# Autodesk Inventor assembly: MGN12H_With_Rail
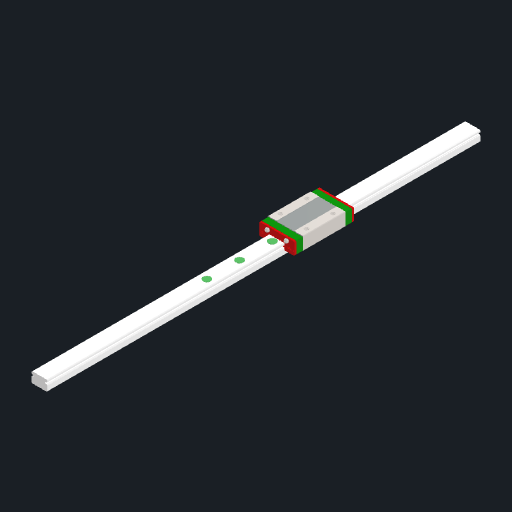
[picture p0: Inventor's stored thumbnail of the model, 512x512]
Saved by Autodesk Inventor 2026.2 (Build 302298000, 298)
## iProperties
Created: 2026-02-12
Part Number: MGN12H_With_Rail
Description: STEP AP214
Document SubType Name: Assembly
Designer: AdminForWorker
Title: MGN12H_With_Rail x axis v1
Author: AdminForWorker
## Documents named in this file (5)
- C:\Users\Alvin\OneDrive\Documents\Inventor\NCKU_Automation_Incubator_Microscope\MGN12H_With_Rail x axis\MGN12H_With_Rail x axis.iam
- C:\Users\Alvin\OneDrive\Documents\Inventor\NCKU_Automation_Incubator_Microscope\MGN12H_With_Rail x axis\MGNR12R100HM.ipt
- C:\Users\Alvin\OneDrive\Documents\Inventor\NCKU_Automation_Incubator_Microscope\MGN12H_With_Rail x axis\MGN12H.iam
- C:\Users\Alvin\OneDrive\Documents\Inventor\NCKU_Automation_Incubator_Microscope\MGN12H_With_Rail x axis\Screw_DIN_912_M3x8F_A2.ipt
- C:\Users\Alvin\OneDrive\Documents\Inventor\NCKU_Automation_Incubator_Microscope\MGN12H_With_Rail x axis\MGN12R_CoverCap.ipt
## Components (10 placed, 4 different names)
1. MGNR12R100HM:1 — Slider:1, Mate:1, Mate:2, Mate:3, Mate:4, Mate:5
2. MGN12H:1 [sub-assembly] — Slider:1, Mate:1, Mate:2, Mate:3, Mate:4, Mate:5
3. Screw_DIN_912_M3x8F_A2:1
4. MGN12R_CoverCap:1
5. Screw_DIN_912_M3x8F_A2:2
6. Screw_DIN_912_M3x8F_A2:3
7. Screw_DIN_912_M3x8F_A2:4
8. MGN12R_CoverCap:2
9. MGN12R_CoverCap:3
10. MGN12R_CoverCap:4
## Relationships (6: Mate 5, TranslationJoint 1)
- Slider:1 [TranslationJoint]: MGNR12R100HM:1 ↔ MGN12H:1
- Mate:1: MGNR12R100HM:1 ↔ MGN12H:1
- Mate:2: MGNR12R100HM:1 ↔ MGN12H:1
- Mate:3: MGNR12R100HM:1 ↔ MGN12H:1
- Mate:4: MGNR12R100HM:1 ↔ MGN12H:1
- Mate:5: MGNR12R100HM:1 ↔ MGN12H:1
